# Autodesk Inventor assembly: Head
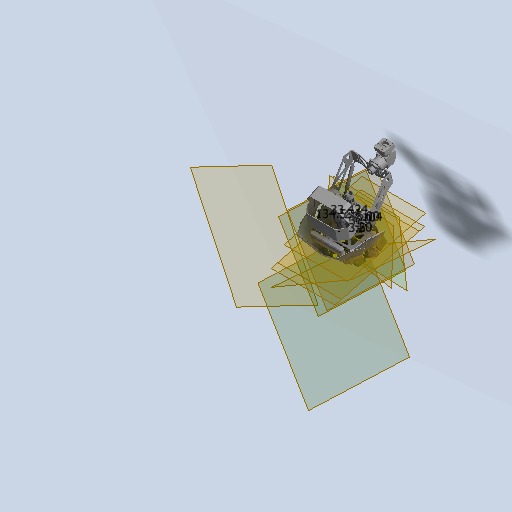
[picture p0: Inventor's stored thumbnail of the model, 512x512]
Saved by Autodesk Inventor 2025.2 (Build 292293000, 293)
## iProperties
Created: 2024-12-17
Part Number: Head
Document SubType Name: Assembly
Designer: valer
Author: valer
## Documents named in this file (46)
- D:\str1ker\cad\Head.iam
- D:\str1ker\cad\Head.ipt
- D:\str1ker\cad\HeadMount.ipt
- D:\str1ker\cad\external\DepthSensor\PrimeSenseCarmine1.09.ipt
- D:\str1ker\cad\external\HingedThreadedStandoffPart1.ipt
- D:\str1ker\cad\external\HingedThreadedStandoffPart2.ipt
- D:\str1ker\cad\ShaftD6FemaleCollar.ipt
- D:\str1ker\cad\external\ShaftD6-2101-0006-0160.ipt
- D:\str1ker\cad\TongueMount.ipt
- D:\str1ker\cad\external\SetScrewLiteHub-1308-0016-0006.ipt
- D:\str1ker\cad\external\ShaftD6-Short-2101-0006-0020.ipt
- D:\str1ker\cad\external\UJoint6D\UJoint6D-Body-4003-1006-1006.ipt
- D:\str1ker\cad\external\UJoint6D\UJoint6D-Screw.ipt
- D:\str1ker\cad\external\ShaftD6-2100-0006-0200.ipt
- D:\str1ker\cad\external\ShaftD6-2101-0006-0140.ipt
- D:\str1ker\cad\external\LinearBearing-1612-0612-0035.ipt
- D:\str1ker\cad\external\ClampingHub1301-0016-0012.ipt
- D:\str1ker\cad\external\ShaftClamp6-6058N14.ipt
- D:\str1ker\cad\external\TongueSpeaker.ipt
- D:\str1ker\cad\TongueSideLid.ipt
- D:\str1ker\cad\TongueSideLidMirror.ipt
- D:\str1ker\cad\NoseMount.ipt
- D:\str1ker\cad\JawMount.ipt
- D:\str1ker\cad\external\93655A703_Male-Female Threaded Hex Standoff.ipt
- D:\str1ker\cad\CameraMount.ipt
- D:\str1ker\cad\external\ServoHorn-1900-0024-0104.ipt
- D:\str1ker\cad\external\Beam4-1102-0004-0032.ipt
- D:\str1ker\cad\Visor.ipt
- D:\str1ker\cad\NeckBase.ipt
- D:\str1ker\cad\NeckBracket.ipt
- D:\str1ker\cad\NeckBracketMirror.ipt
- D:\str1ker\cad\NeckCover.ipt
- D:\str1ker\cad\external\ArmPotentiometer\rh24pce.iam
- D:\str1ker\cad\NeckMiddleBracket.ipt
- D:\str1ker\cad\external\Max9744_20W_ClassD_Amplifier.ipt
- D:\str1ker\cad\external\ArmDriver\IBTMini.ipt
- D:\str1ker\cad\external\HeadServo\M3RCServoMountBracket.ipt
- D:\str1ker\cad\NeckMount.ipt
- D:\str1ker\cad\external\1611-0514-0006.ipt
- D:\str1ker\cad\external\pololu-universal-aluminum-mounting-hub-for-6mm-shaft-m3-holes.ipt
- D:\str1ker\cad\external\WHITE JST XH 3 PIN CONNECTOR - P 2.54mm - ANGLED.ipt
- D:\str1ker\cad\external\NeckActuator\1610-50H-2KG-12V-B07-Body.ipt
- D:\str1ker\cad\external\NeckActuator\1610-50H-2KG-12V-B07-Shaft.ipt
- D:\str1ker\cad\external\59935K12_Ball Joint Rod End.ipt
- D:\str1ker\cad\external\RYG23-G10-D8.iam
- D:\str1ker\cad\external\NexusRobot14mmKeywayHub.ipt
## Components (95 placed, 45 different names)
1. Head:1 — Flush:1, Flush:2, Mate:1, Flush:3, Mate:4, Mate:5, Mate:6, Mate:7, Mate:8, Mate:9, Mate:10, Mate:11, Mate:12, Mate:13, Mate:14, Mate:15, Mate:16, Mate:17, Mate:18, Mate:19, Mate:20, Mate:59, Angle:13, Mate:89, Mate:90, Flush:13, Mate:119, Mate:121, Flush:15, Flush:16, Flush:17, Flush:18, Flush:19, Mate:124, Mate:125, Mate:126, Mate:127, Mate:128, Mate:129, Flush:20, Mate:131, Mate:132, Mate:133, Flush:157, Flush:166, Mate:230
2. HeadMount:1 — Flush:4, Flush:5, Angle:18, Mate:89, Mate:90, Angle:20, Angle:22, Angle:26, Angle:28, Angle:32, Mate:105, Mate:107, Mate:109, Mate:111, Mate:113, Mate:115, Mate:134, Mate:135, Mate:136, Mate:137, Flush:158, Mate:178, Angle:37, Mate:293, Mate:299, Mate:308, Mate:309, Mate:311, Mate:312, Mate:344, Mate:347, Flush:181, Mate:376, Mate:377, Mate:384, Mate:387
3. PrimeSenseCarmine1.09:1 — Flush:6, Flush:23, Mate:138, Mate:198
4. HingedThreadedStandoffPart1:1 — Mate:4, Mate:5, Mate:25, Mate:26
5. HingedThreadedStandoffPart1:2 — Mate:6, Mate:7, Mate:36, Mate:39
6. HingedThreadedStandoffPart1:3 — Mate:8, Mate:9, Mate:37, Mate:38
7. HingedThreadedStandoffPart1:4 — Mate:10, Mate:11, Mate:23, Mate:24
8. HingedThreadedStandoffPart1:5 — Mate:12, Mate:13, Mate:27, Mate:28
9. HingedThreadedStandoffPart1:6 — Mate:16, Mate:17, Mate:29, Mate:40
10. HingedThreadedStandoffPart1:7 — Mate:14, Mate:15, Mate:30, Mate:31
11. HingedThreadedStandoffPart1:8 — Mate:18, Mate:19, Mate:32, Mate:34
12. HingedThreadedStandoffPart1:9 — Mate:20, Mate:33, Mate:35, Mate:59
13. HingedThreadedStandoffPart2:4 — Mate:23, Mate:24, Flush:7, Flush:8
14. HingedThreadedStandoffPart2:5 — Mate:25, Mate:26, Flush:8, Mate:68
15. HingedThreadedStandoffPart2:6 — Mate:27, Mate:28, Flush:7, Flush:10, Mate:69
16. HingedThreadedStandoffPart2:7 — Mate:29, Mate:40, Mate:45, Mate:47
17. HingedThreadedStandoffPart2:8 — Mate:30, Mate:31, Mate:46, Mate:48
18. HingedThreadedStandoffPart2:9 — Mate:32, Mate:34, Mate:49, Mate:52
19. HingedThreadedStandoffPart2:10 — Mate:33, Mate:35, Mate:50, Mate:51
20. HingedThreadedStandoffPart2:11 — Mate:36, Mate:39, Mate:41, Mate:42
21. HingedThreadedStandoffPart2:12 — Mate:37, Mate:38, Mate:43, Mate:44
22. ShaftD6-2100-0006-0200:1 — Mate:87, Angle:17, Mate:88, Angle:18, Mate:108
23. ShaftD6FemaleCollar:1 — Mate:41, Mate:42, Mate:87, Angle:17, Mate:88
24. ShaftD6FemaleCollar:2 — Mate:43, Mate:44, Mate:91, Mate:92
25. ShaftD6FemaleCollar:3 — Mate:45, Mate:47, Mate:95, Mate:96, Angle:23
26. ShaftD6FemaleCollar:4 — Mate:46, Mate:48, Mate:93, Mate:94, Angle:21
27. ShaftD6FemaleCollar:5 — Mate:49, Mate:52, Mate:99, Mate:100, Angle:30
28. ShaftD6FemaleCollar:6 — Mate:50, Mate:51, Mate:97, Mate:98, Angle:27
29. TongueMount:1 — Mate:66, Mate:67, Angle:11, Mate:68, Mate:69, Mate:71
30. SetScrewLiteHub-1308-0016-0006:1 — Mate:66, Mate:67, Angle:11, Mate:70, Mate:73
31. ShaftD6-Short-2101-0006-0020:1 — Mate:70, Mate:71, Mate:72, Angle:12
32. UJoint6D-Body-4003-1006-1006:1 — Mate:72, Mate:73, Angle:12, Mate:76, Mate:77, Mate:78, Mate:79
33. UJoint6D-Screw:1 — Mate:82, Mate:83
34. UJoint6D-Screw:2 — Mate:76, Mate:77
35. UJoint6D-Screw:3 — Mate:78, Mate:79
36. UJoint6D-Body-4003-1006-1006:2 — Angle:13, Mate:82, Mate:83, Mate:84, Mate:85, Mate:86, Angle:14, Flush:12
37. UJoint6D-Screw:4 — Mate:84, Mate:85
38. ShaftD6-2101-0006-0160:7 — Mate:86, Angle:14, Flush:12, Mate:101, Mate:168, Flush:184
39. ShaftD6-2100-0006-0200:2 — Mate:91, Mate:92, Angle:19, Angle:20, Mate:110
40. ShaftD6-2101-0006-0140:1 — Mate:93, Mate:94, Angle:21, Angle:22, Angle:24, Mate:104
41. ShaftD6-2101-0006-0140:2 — Mate:95, Mate:96, Angle:23, Angle:25, Angle:26, Mate:106
42. ShaftD6-2101-0006-0140:3 — Mate:97, Mate:98, Angle:27, Angle:28, Angle:29, Mate:112
43. ShaftD6-2101-0006-0140:4 — Mate:99, Mate:100, Angle:30, Angle:31, Angle:32, Mate:114
44. LinearBearing-1612-0612-0035:1 — Mate:101, Mate:103, Flush:160
45. ClampingHub1301-0016-0012:1 — Mate:103, Flush:160, Angle:37, Mate:347
46. ShaftClamp6-6058N14:1 — Mate:106, Mate:107
47. ShaftClamp6-6058N14:2 — Mate:104, Mate:105
48. ShaftClamp6-6058N14:3 — Mate:108, Mate:109
49. ShaftClamp6-6058N14:4 — Mate:110, Mate:111
50. ShaftClamp6-6058N14:5 — Mate:114, Mate:115
51. ShaftClamp6-6058N14:6 — Mate:112, Mate:113
52. TongueSpeaker:1 — Mate:119, Mate:122, Mate:123
53. TongueSpeaker:2 — Mate:121, Mate:130
54. TongueSideLid:1 — Mate:124, Mate:125, Mate:126
55. TongueSideLidMirror:1 — Mate:127, Mate:128, Mate:129, Mate:130
56. NoseMount:1 — Flush:21, Mate:131, Mate:132, Mate:133
57. JawMount:1 — Flush:22
58. 93655A703_Male-Female Threaded Hex Standoff:1 — Mate:134, Mate:136, Mate:141, Mate:143
59. 93655A703_Male-Female Threaded Hex Standoff:2 — Mate:135, Mate:137, Mate:142
60. CameraMount:1 — Flush:24, Mate:138, Mate:141, Mate:142, Mate:143, Mate:198
61. ShaftClamp6-6058N14:8 — Mate:168, Flush:184
62. Visor:1 — Flush:157, Flush:158, Mate:178
63. NeckBracket:1 — Mate:239, Mate:240, Mate:241, Mate:244, Mate:286, Mate:392
64. NeckCover:1 — Flush:166, Mate:353, Mate:354
65. NeckCover:2 — Mate:244, Mate:250, Mate:251, Mate:354
66. NeckMiddleBracket:1 — Mate:230, Flush:172, Flush:173, Mate:273, Mate:286, Mate:329, Angle:52, Mate:352, Flush:182
67. NeckBase:1 — Mate:239, Mate:240, Mate:241, Mate:246, Mate:247, Mate:248, Angle:55, Mate:395, Mate:396, Mate:397
68. NeckBracketMirror:1 — Mate:246, Mate:247, Mate:248, Mate:250, Mate:251, Flush:172, Flush:173, Mate:353, Mate:381
69. IBTMini:1 — Mate:273, Mate:352, Flush:182
70. NeckMount:1 — Mate:310, Flush:177, Mate:317, Mate:318, Mate:328, Mate:330, Mate:340, Mate:341
71. NeckMount:2 — Mate:313, Flush:177, Mate:319, Mate:320, Mate:326, Mate:329, Mate:334
72. 1611-0514-0006:1 — Mate:319, Mate:320
73. 1611-0514-0006:2 — Mate:314, Mate:315, Mate:336
74. NeckMount:3 — Mate:293, Mate:308, Mate:310, Mate:311, Mate:314, Mate:315, Mate:328, Mate:337, Mate:338
75. NeckMount:4 — Mate:299, Mate:309, Mate:312, Mate:313, Mate:316, Mate:326, Mate:346
76. 1611-0514-0006:4 — Mate:316
77. WHITE JST XH 3 PIN CONNECTOR - P 2.54mm - ANGLED:1 — Flush:179, Mate:333, Flush:180, Angle:52
78. rh24pce:1 [sub-assembly] — Mate:330, Flush:179, Mate:333, Flush:180, Mate:334
79. 1611-0514-0006:5 — Mate:317, Mate:318, Mate:339
80. M3RCServoMountBracket:1 — Mate:344, Mate:346, Flush:181
81. ServoHorn-1900-0024-0104:1 — Mate:350, Mate:351
82. Beam4-1102-0004-0032:1 — Mate:350, Mate:351
83. Max9744_20W_ClassD_Amplifier:1
84. pololu-universal-aluminum-mounting-hub-for-6mm-shaft-m3-holes:4 — Mate:339, Mate:340, Mate:341
85. pololu-universal-aluminum-mounting-hub-for-6mm-shaft-m3-holes:5 — Mate:336, Mate:337, Mate:338
86. 1610-50H-2KG-12V-B07-Body:1 — Cylindrical:1, Mate:378, Mate:379, Mate:383
87. 1610-50H-2KG-12V-B07-Shaft:1 — Cylindrical:1, Mate:380, Mate:382, Mate:383
88. 1610-50H-2KG-12V-B07-Body:2 — Mate:385, Mate:386, Mate:390, Mate:391
89. 59935K12_Ball Joint Rod End:1 — Mate:378, Mate:379, Mate:381
90. 59935K12_Ball Joint Rod End:2 — Mate:385, Mate:386, Mate:392
91. 59935K12_Ball Joint Rod End:3 — Mate:376, Mate:380, Mate:382, Mate:384
92. 59935K12_Ball Joint Rod End:4 — Mate:377, Mate:387, Mate:388, Mate:389
93. 1610-50H-2KG-12V-B07-Shaft:2 — Mate:388, Mate:389, Mate:390, Mate:391
94. RYG23-G10-D8:1 [sub-assembly] — Mate:394, Angle:55, Mate:398
95. NexusRobot14mmKeywayHub:1 — Mate:394, Mate:395, Mate:396, Mate:397, Mate:398
## Relationships (248: Mate 189, Flush 33, Angle 23, Symmetry 2, CylindricalJoint 1)
- Flush:1: Head:1
- Flush:2: Head:1
- Mate:1: Head:1
- Flush:3: Head:1
- Flush:4: HeadMount:1
- Flush:5: HeadMount:1
- Flush:6: PrimeSenseCarmine1.09:1
- Mate:4: Head:1 ↔ HingedThreadedStandoffPart1:1
- Mate:5: Head:1 ↔ HingedThreadedStandoffPart1:1
- Mate:6: Head:1 ↔ HingedThreadedStandoffPart1:2
- Mate:7: Head:1 ↔ HingedThreadedStandoffPart1:2
- Mate:8: Head:1 ↔ HingedThreadedStandoffPart1:3
- Mate:9: Head:1 ↔ HingedThreadedStandoffPart1:3
- Mate:10: Head:1 ↔ HingedThreadedStandoffPart1:4
- Mate:11: Head:1 ↔ HingedThreadedStandoffPart1:4
- Mate:12: Head:1 ↔ HingedThreadedStandoffPart1:5
- Mate:13: Head:1 ↔ HingedThreadedStandoffPart1:5
- Mate:14: Head:1 ↔ HingedThreadedStandoffPart1:7
- Mate:15: Head:1 ↔ HingedThreadedStandoffPart1:7
- Mate:16: Head:1 ↔ HingedThreadedStandoffPart1:6
- Mate:17: Head:1 ↔ HingedThreadedStandoffPart1:6
- Mate:18: Head:1 ↔ HingedThreadedStandoffPart1:8
- Mate:19: Head:1 ↔ HingedThreadedStandoffPart1:8
- Mate:20: Head:1 ↔ HingedThreadedStandoffPart1:9
- Mate:23: HingedThreadedStandoffPart1:4 ↔ HingedThreadedStandoffPart2:4
- Mate:24: HingedThreadedStandoffPart1:4 ↔ HingedThreadedStandoffPart2:4
- Mate:25: HingedThreadedStandoffPart1:1 ↔ HingedThreadedStandoffPart2:5
- Mate:26: HingedThreadedStandoffPart1:1 ↔ HingedThreadedStandoffPart2:5
- Mate:27: HingedThreadedStandoffPart1:5 ↔ HingedThreadedStandoffPart2:6
- Mate:28: HingedThreadedStandoffPart1:5 ↔ HingedThreadedStandoffPart2:6
- Mate:29: HingedThreadedStandoffPart1:6 ↔ HingedThreadedStandoffPart2:7
- Mate:30: HingedThreadedStandoffPart1:7 ↔ HingedThreadedStandoffPart2:8
- Mate:31: HingedThreadedStandoffPart1:7 ↔ HingedThreadedStandoffPart2:8
- Mate:32: HingedThreadedStandoffPart1:8 ↔ HingedThreadedStandoffPart2:9
- Mate:33: HingedThreadedStandoffPart1:9 ↔ HingedThreadedStandoffPart2:10
- Mate:34: HingedThreadedStandoffPart1:8 ↔ HingedThreadedStandoffPart2:9
- Mate:35: HingedThreadedStandoffPart1:9 ↔ HingedThreadedStandoffPart2:10
- Mate:36: HingedThreadedStandoffPart1:2 ↔ HingedThreadedStandoffPart2:11
- Mate:37: HingedThreadedStandoffPart1:3 ↔ HingedThreadedStandoffPart2:12
- Mate:38: HingedThreadedStandoffPart1:3 ↔ HingedThreadedStandoffPart2:12
- Mate:39: HingedThreadedStandoffPart1:2 ↔ HingedThreadedStandoffPart2:11
- Mate:40: HingedThreadedStandoffPart1:6 ↔ HingedThreadedStandoffPart2:7
- Flush:7: HingedThreadedStandoffPart2:4 ↔ HingedThreadedStandoffPart2:6
- Flush:8: HingedThreadedStandoffPart2:4 ↔ HingedThreadedStandoffPart2:5
- Mate:41: HingedThreadedStandoffPart2:11 ↔ ShaftD6FemaleCollar:1
- Mate:42: HingedThreadedStandoffPart2:11 ↔ ShaftD6FemaleCollar:1
- Mate:43: HingedThreadedStandoffPart2:12 ↔ ShaftD6FemaleCollar:2
- Mate:44: HingedThreadedStandoffPart2:12 ↔ ShaftD6FemaleCollar:2
- Mate:45: HingedThreadedStandoffPart2:7 ↔ ShaftD6FemaleCollar:3
- Mate:46: HingedThreadedStandoffPart2:8 ↔ ShaftD6FemaleCollar:4
- Mate:47: HingedThreadedStandoffPart2:7 ↔ ShaftD6FemaleCollar:3
- Mate:48: HingedThreadedStandoffPart2:8 ↔ ShaftD6FemaleCollar:4
- Mate:49: HingedThreadedStandoffPart2:9 ↔ ShaftD6FemaleCollar:5
- Mate:50: HingedThreadedStandoffPart2:10 ↔ ShaftD6FemaleCollar:6
- Mate:51: HingedThreadedStandoffPart2:10 ↔ ShaftD6FemaleCollar:6
- Mate:52: HingedThreadedStandoffPart2:9 ↔ ShaftD6FemaleCollar:5
- Mate:59: Head:1 ↔ HingedThreadedStandoffPart1:9
- Flush:10: HingedThreadedStandoffPart2:6
- Mate:66: TongueMount:1 ↔ SetScrewLiteHub-1308-0016-0006:1
- Mate:67: TongueMount:1 ↔ SetScrewLiteHub-1308-0016-0006:1
- Angle:11 (0 deg): TongueMount:1 ↔ SetScrewLiteHub-1308-0016-0006:1
- Mate:68: HingedThreadedStandoffPart2:5 ↔ TongueMount:1
- Mate:69: HingedThreadedStandoffPart2:6 ↔ TongueMount:1
- Mate:70: SetScrewLiteHub-1308-0016-0006:1 ↔ ShaftD6-Short-2101-0006-0020:1
- Mate:71: TongueMount:1 ↔ ShaftD6-Short-2101-0006-0020:1
- Mate:72: ShaftD6-Short-2101-0006-0020:1 ↔ UJoint6D-Body-4003-1006-1006:1
- Mate:73: SetScrewLiteHub-1308-0016-0006:1 ↔ UJoint6D-Body-4003-1006-1006:1
- Angle:12 (0 deg): ShaftD6-Short-2101-0006-0020:1 ↔ UJoint6D-Body-4003-1006-1006:1
- Mate:76: UJoint6D-Body-4003-1006-1006:1 ↔ UJoint6D-Screw:2
- Mate:77: UJoint6D-Body-4003-1006-1006:1 ↔ UJoint6D-Screw:2
- Mate:78: UJoint6D-Body-4003-1006-1006:1 ↔ UJoint6D-Screw:3
- Mate:79: UJoint6D-Body-4003-1006-1006:1 ↔ UJoint6D-Screw:3
- Angle:13 (0 deg): Head:1 ↔ UJoint6D-Body-4003-1006-1006:2
- Mate:82: UJoint6D-Screw:1 ↔ UJoint6D-Body-4003-1006-1006:2
- Mate:83: UJoint6D-Screw:1 ↔ UJoint6D-Body-4003-1006-1006:2
- Mate:84: UJoint6D-Body-4003-1006-1006:2 ↔ UJoint6D-Screw:4
- Mate:85: UJoint6D-Body-4003-1006-1006:2 ↔ UJoint6D-Screw:4
- Mate:86: UJoint6D-Body-4003-1006-1006:2 ↔ ShaftD6-2101-0006-0160:7
- Angle:14 (180 deg): UJoint6D-Body-4003-1006-1006:2 ↔ ShaftD6-2101-0006-0160:7
- Flush:12: UJoint6D-Body-4003-1006-1006:2 ↔ ShaftD6-2101-0006-0160:7
- Mate:87: ShaftD6-2100-0006-0200:1 ↔ ShaftD6FemaleCollar:1
- Angle:17 (0 deg): ShaftD6-2100-0006-0200:1 ↔ ShaftD6FemaleCollar:1
- Mate:88: ShaftD6-2100-0006-0200:1 ↔ ShaftD6FemaleCollar:1
- Angle:18 (0 deg): HeadMount:1 ↔ ShaftD6-2100-0006-0200:1
- Mate:89: Head:1 ↔ HeadMount:1
- Mate:90: Head:1 ↔ HeadMount:1
- Mate:91: ShaftD6FemaleCollar:2 ↔ ShaftD6-2100-0006-0200:2
- Mate:92: ShaftD6FemaleCollar:2 ↔ ShaftD6-2100-0006-0200:2
- Angle:19 (0 deg): ShaftD6-2100-0006-0200:2
- Angle:20 (0 deg): HeadMount:1 ↔ ShaftD6-2100-0006-0200:2
- Mate:93: ShaftD6FemaleCollar:4 ↔ ShaftD6-2101-0006-0140:1
- Mate:94: ShaftD6FemaleCollar:4 ↔ ShaftD6-2101-0006-0140:1
- Angle:21 (0 deg): ShaftD6FemaleCollar:4 ↔ ShaftD6-2101-0006-0140:1
- Angle:22 (0 deg): HeadMount:1 ↔ ShaftD6-2101-0006-0140:1
- Mate:95: ShaftD6FemaleCollar:3 ↔ ShaftD6-2101-0006-0140:2
- Mate:96: ShaftD6FemaleCollar:3 ↔ ShaftD6-2101-0006-0140:2
- Angle:23 (0 deg): ShaftD6FemaleCollar:3 ↔ ShaftD6-2101-0006-0140:2
- Angle:24 (180 deg): ShaftD6-2101-0006-0140:1
- Angle:25 (180 deg): ShaftD6-2101-0006-0140:2
- Angle:26 (0 deg): HeadMount:1 ↔ ShaftD6-2101-0006-0140:2
- Mate:97: ShaftD6FemaleCollar:6 ↔ ShaftD6-2101-0006-0140:3
- Mate:98: ShaftD6FemaleCollar:6 ↔ ShaftD6-2101-0006-0140:3
- Angle:27 (0 deg): ShaftD6FemaleCollar:6 ↔ ShaftD6-2101-0006-0140:3
- Angle:28 (0 deg): HeadMount:1 ↔ ShaftD6-2101-0006-0140:3
- Angle:29 (0 deg): ShaftD6-2101-0006-0140:3
- Mate:99: ShaftD6FemaleCollar:5 ↔ ShaftD6-2101-0006-0140:4
- Mate:100: ShaftD6FemaleCollar:5 ↔ ShaftD6-2101-0006-0140:4
- Angle:30 (0 deg): ShaftD6FemaleCollar:5 ↔ ShaftD6-2101-0006-0140:4
- Angle:31 (0 deg): ShaftD6-2101-0006-0140:4
- Angle:32 (0 deg): HeadMount:1 ↔ ShaftD6-2101-0006-0140:4
- Mate:101: ShaftD6-2101-0006-0160:7 ↔ LinearBearing-1612-0612-0035:1
- Mate:103: LinearBearing-1612-0612-0035:1 ↔ ClampingHub1301-0016-0012:1
- Mate:104: ShaftD6-2101-0006-0140:1 ↔ ShaftClamp6-6058N14:2
- Mate:105: HeadMount:1 ↔ ShaftClamp6-6058N14:2
- Mate:106: ShaftD6-2101-0006-0140:2 ↔ ShaftClamp6-6058N14:1
- Mate:107: HeadMount:1 ↔ ShaftClamp6-6058N14:1
- Mate:108: ShaftD6-2100-0006-0200:1 ↔ ShaftClamp6-6058N14:3
- Mate:109: HeadMount:1 ↔ ShaftClamp6-6058N14:3
- Mate:110: ShaftD6-2100-0006-0200:2 ↔ ShaftClamp6-6058N14:4
- Mate:111: HeadMount:1 ↔ ShaftClamp6-6058N14:4
- Mate:112: ShaftD6-2101-0006-0140:3 ↔ ShaftClamp6-6058N14:6
- Mate:113: HeadMount:1 ↔ ShaftClamp6-6058N14:6
- Mate:114: ShaftD6-2101-0006-0140:4 ↔ ShaftClamp6-6058N14:5
- Mate:115: HeadMount:1 ↔ ShaftClamp6-6058N14:5
- Flush:13: Head:1
- Mate:119: Head:1 ↔ TongueSpeaker:1
- Mate:121: Head:1 ↔ TongueSpeaker:2
- Flush:15: Head:1
- Flush:16: Head:1
- Symmetry:1
- Mate:122: TongueSpeaker:1
- Flush:17: Head:1
- Flush:18: Head:1
- Symmetry:2
- Mate:123: TongueSpeaker:1
- Flush:19: Head:1
- Mate:124: Head:1 ↔ TongueSideLid:1
- Mate:125: Head:1 ↔ TongueSideLid:1
- Mate:126: Head:1 ↔ TongueSideLid:1
- Mate:127: Head:1 ↔ TongueSideLidMirror:1
- Mate:128: Head:1 ↔ TongueSideLidMirror:1
- Mate:129: Head:1 ↔ TongueSideLidMirror:1
- Mate:130: TongueSpeaker:2 ↔ TongueSideLidMirror:1
- Flush:20: Head:1
- Flush:21: NoseMount:1
- Mate:131: Head:1 ↔ NoseMount:1
- Mate:132: Head:1 ↔ NoseMount:1
- Mate:133: Head:1 ↔ NoseMount:1
- Flush:22: JawMount:1
- Mate:134: HeadMount:1 ↔ 93655A703_Male-Female Threaded Hex Standoff:1
- Mate:135: HeadMount:1 ↔ 93655A703_Male-Female Threaded Hex Standoff:2
- Mate:136: HeadMount:1 ↔ 93655A703_Male-Female Threaded Hex Standoff:1
- Mate:137: HeadMount:1 ↔ 93655A703_Male-Female Threaded Hex Standoff:2
- Flush:23: PrimeSenseCarmine1.09:1
- Flush:24: CameraMount:1
- Mate:138: PrimeSenseCarmine1.09:1 ↔ CameraMount:1
- Mate:141: 93655A703_Male-Female Threaded Hex Standoff:1 ↔ CameraMount:1
- Mate:142: 93655A703_Male-Female Threaded Hex Standoff:2 ↔ CameraMount:1
- Mate:143: 93655A703_Male-Female Threaded Hex Standoff:1 ↔ CameraMount:1
- Mate:168: ShaftD6-2101-0006-0160:7 ↔ ShaftClamp6-6058N14:8
- Flush:157: Head:1 ↔ Visor:1
- Flush:158: HeadMount:1 ↔ Visor:1
- Mate:178: HeadMount:1 ↔ Visor:1
- Flush:160: LinearBearing-1612-0612-0035:1 ↔ ClampingHub1301-0016-0012:1
- Mate:198: PrimeSenseCarmine1.09:1 ↔ CameraMount:1
- Angle:37 (0 deg): HeadMount:1 ↔ ClampingHub1301-0016-0012:1
- Flush:166: Head:1 ↔ NeckCover:1
- Mate:230: Head:1 ↔ NeckMiddleBracket:1
- Mate:239: NeckBracket:1 ↔ NeckBase:1
- Mate:240: NeckBracket:1 ↔ NeckBase:1
- Mate:241: NeckBracket:1 ↔ NeckBase:1
- Mate:244: NeckBracket:1 ↔ NeckCover:2
- Mate:246: NeckBase:1 ↔ NeckBracketMirror:1
- Mate:247: NeckBase:1 ↔ NeckBracketMirror:1
- Mate:248: NeckBase:1 ↔ NeckBracketMirror:1
- Mate:250: NeckCover:2 ↔ NeckBracketMirror:1
- Mate:251: NeckCover:2 ↔ NeckBracketMirror:1
- Flush:172: NeckMiddleBracket:1 ↔ NeckBracketMirror:1
- Flush:173: NeckMiddleBracket:1 ↔ NeckBracketMirror:1
- Mate:273: NeckMiddleBracket:1 ↔ IBTMini:1
- Mate:286: NeckBracket:1 ↔ NeckMiddleBracket:1
- Mate:293: HeadMount:1 ↔ NeckMount:3
- [Mate]: NeckMount:4 ↔ 1611-0514-0006:4
- Mate:299: HeadMount:1 ↔ NeckMount:4
- Mate:308: HeadMount:1 ↔ NeckMount:3
- Mate:309: HeadMount:1 ↔ NeckMount:4
- Mate:310: NeckMount:1 ↔ NeckMount:3
- Mate:311: HeadMount:1 ↔ NeckMount:3
- Mate:312: HeadMount:1 ↔ NeckMount:4
- Mate:313: NeckMount:2 ↔ NeckMount:4
- Flush:177: NeckMount:1 ↔ NeckMount:2
- Mate:314: 1611-0514-0006:2 ↔ NeckMount:3
- Mate:315: 1611-0514-0006:2 ↔ NeckMount:3
- Mate:316: NeckMount:4 ↔ 1611-0514-0006:4
- Mate:317: NeckMount:1 ↔ 1611-0514-0006:5
- Mate:318: NeckMount:1 ↔ 1611-0514-0006:5
- Mate:319: NeckMount:2 ↔ 1611-0514-0006:1
- Mate:320: NeckMount:2 ↔ 1611-0514-0006:1
- Mate:326: NeckMount:2 ↔ NeckMount:4
- Mate:328: NeckMount:1 ↔ NeckMount:3
- Mate:329: NeckMiddleBracket:1 ↔ NeckMount:2
- Mate:330: NeckMount:1 ↔ rh24pce:1
- Flush:179 (6.15 mm): WHITE JST XH 3 PIN CONNECTOR - P 2.54mm - ANGLED:1 ↔ rh24pce:1
- Mate:333: WHITE JST XH 3 PIN CONNECTOR - P 2.54mm - ANGLED:1 ↔ rh24pce:1
- Flush:180: WHITE JST XH 3 PIN CONNECTOR - P 2.54mm - ANGLED:1 ↔ rh24pce:1
- Angle:52 (0 deg): NeckMiddleBracket:1 ↔ WHITE JST XH 3 PIN CONNECTOR - P 2.54mm - ANGLED:1
- Mate:334: NeckMount:2 ↔ rh24pce:1
- Mate:336: 1611-0514-0006:2 ↔ pololu-universal-aluminum-mounting-hub-for-6mm-shaft-m3-holes:5
- Mate:337: NeckMount:3 ↔ pololu-universal-aluminum-mounting-hub-for-6mm-shaft-m3-holes:5
- Mate:338: NeckMount:3 ↔ pololu-universal-aluminum-mounting-hub-for-6mm-shaft-m3-holes:5
- Mate:339: 1611-0514-0006:5 ↔ pololu-universal-aluminum-mounting-hub-for-6mm-shaft-m3-holes:4
- Mate:340: NeckMount:1 ↔ pololu-universal-aluminum-mounting-hub-for-6mm-shaft-m3-holes:4
- Mate:341: NeckMount:1 ↔ pololu-universal-aluminum-mounting-hub-for-6mm-shaft-m3-holes:4
- Mate:344: HeadMount:1 ↔ M3RCServoMountBracket:1
- Mate:346: NeckMount:4 ↔ M3RCServoMountBracket:1
- Mate:347: HeadMount:1 ↔ ClampingHub1301-0016-0012:1
- Flush:181: HeadMount:1 ↔ M3RCServoMountBracket:1
- Mate:350: ServoHorn-1900-0024-0104:1 ↔ Beam4-1102-0004-0032:1
- Mate:351: ServoHorn-1900-0024-0104:1 ↔ Beam4-1102-0004-0032:1
- Mate:352: NeckMiddleBracket:1 ↔ IBTMini:1
- Flush:182: NeckMiddleBracket:1 ↔ IBTMini:1
- Mate:353: NeckCover:1 ↔ NeckBracketMirror:1
- Mate:354: NeckCover:1 ↔ NeckCover:2
- Mate:376: HeadMount:1 ↔ 59935K12_Ball Joint Rod End:3
- Mate:377: HeadMount:1 ↔ 59935K12_Ball Joint Rod End:4
- Cylindrical:1: 1610-50H-2KG-12V-B07-Body:1 ↔ 1610-50H-2KG-12V-B07-Shaft:1
- Mate:378: 1610-50H-2KG-12V-B07-Body:1 ↔ 59935K12_Ball Joint Rod End:1
- Mate:379: 1610-50H-2KG-12V-B07-Body:1 ↔ 59935K12_Ball Joint Rod End:1
- Mate:380: 1610-50H-2KG-12V-B07-Shaft:1 ↔ 59935K12_Ball Joint Rod End:3
- Mate:381: NeckBracketMirror:1 ↔ 59935K12_Ball Joint Rod End:1
- Mate:382: 1610-50H-2KG-12V-B07-Shaft:1 ↔ 59935K12_Ball Joint Rod End:3
- Mate:383: 1610-50H-2KG-12V-B07-Body:1 ↔ 1610-50H-2KG-12V-B07-Shaft:1
- Mate:384 (8 mm): HeadMount:1 ↔ 59935K12_Ball Joint Rod End:3
- Flush:184: ShaftD6-2101-0006-0160:7 ↔ ShaftClamp6-6058N14:8
- Mate:385: 1610-50H-2KG-12V-B07-Body:2 ↔ 59935K12_Ball Joint Rod End:2
- Mate:386: 1610-50H-2KG-12V-B07-Body:2 ↔ 59935K12_Ball Joint Rod End:2
- Mate:387 (8 mm): HeadMount:1 ↔ 59935K12_Ball Joint Rod End:4
- Mate:388: 59935K12_Ball Joint Rod End:4 ↔ 1610-50H-2KG-12V-B07-Shaft:2
- Mate:389: 59935K12_Ball Joint Rod End:4 ↔ 1610-50H-2KG-12V-B07-Shaft:2
- Mate:390: 1610-50H-2KG-12V-B07-Body:2 ↔ 1610-50H-2KG-12V-B07-Shaft:2
- Mate:391: 1610-50H-2KG-12V-B07-Body:2 ↔ 1610-50H-2KG-12V-B07-Shaft:2
- Mate:392: NeckBracket:1 ↔ 59935K12_Ball Joint Rod End:2
- Mate:394: RYG23-G10-D8:1 ↔ NexusRobot14mmKeywayHub:1
- Angle:55 (0 deg): NeckBase:1 ↔ RYG23-G10-D8:1
- Mate:395: NeckBase:1 ↔ NexusRobot14mmKeywayHub:1
- Mate:396: NeckBase:1 ↔ NexusRobot14mmKeywayHub:1
- Mate:397: NeckBase:1 ↔ NexusRobot14mmKeywayHub:1
- Mate:398: RYG23-G10-D8:1 ↔ NexusRobot14mmKeywayHub:1
## Named parameters: d567_d562_d558 = 0 mm
